# Autodesk Inventor assembly: 5 Barras Version 0
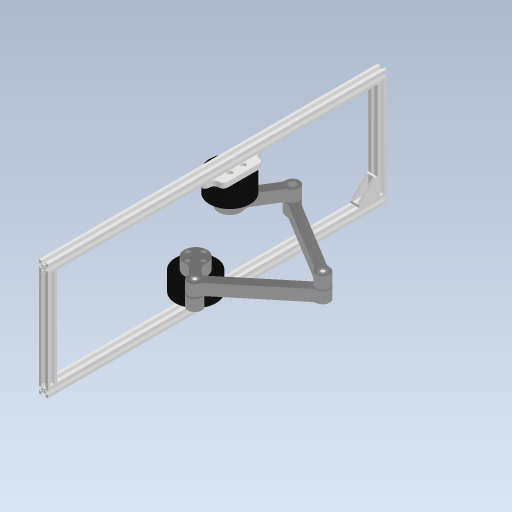
[picture p0: Inventor's stored thumbnail of the model, 512x512]
Saved by Autodesk Inventor 2024.2 (Build 282272000, 272)
## iProperties
Created: 2025-02-06
Part Number: 5 Barras Version 0
Document SubType Name: Assembly
Designer: jp.reyesf
Author: jp.reyesf
## Documents named in this file (18)
- C:\Users\jp.reyesf\Desktop\Master-Thesis\five_bar\assets\CAD\Robot\5 Barras Version 0.iam
- C:\Users\jp.reyesf\Desktop\Master-Thesis\five_bar\assets\CAD\Robot\Proximal Link 1.ipt
- C:\Users\jp.reyesf\Desktop\Master-Thesis\five_bar\assets\CAD\Robot\Distal Link 1.ipt
- C:\Users\jp.reyesf\Desktop\Master-Thesis\five_bar\assets\CAD\Robot\Distal Link 2.ipt
- C:\Users\jp.reyesf\Desktop\Master-Thesis\five_bar\assets\CAD\Robot\Proximal Link 2.ipt
- C:\Users\jp.reyesf\Desktop\Master-Thesis\five_bar\assets\CAD\Robot\Spacer.ipt
- C:\Users\jp.reyesf\Desktop\Master-Thesis\five_bar\assets\CAD\Robot\Bearing.ipt
- C:\Users\jp.reyesf\Desktop\Master-Thesis\five_bar\assets\CAD\Robot\Motor 1 Stator.ipt
- C:\Users\jp.reyesf\Desktop\Master-Thesis\five_bar\assets\CAD\Robot\Motor 1 Rotor.ipt
- C:\Users\jp.reyesf\Desktop\Master-Thesis\five_bar\assets\CAD\Robot\Motor 2 Stator.ipt
- C:\Users\jp.reyesf\Desktop\Master-Thesis\five_bar\assets\CAD\Robot\Motor 2 Rotor.ipt
- C:\Users\jp.reyesf\Desktop\Master-Thesis\five_bar\assets\CAD\Robot\separator.ipt
- C:\Users\jp.reyesf\Desktop\Master-Thesis\five_bar\assets\CAD\Robot\rod.ipt
- C:\Users\jp.reyesf\Desktop\Master-Thesis\five_bar\assets\CAD\Robot\Solid35.ipt
- C:\Users\jp.reyesf\Desktop\Master-Thesis\five_bar\assets\CAD\Robot\Solid37.ipt
- C:\Users\jp.reyesf\Desktop\Master-Thesis\five_bar\assets\CAD\Robot\Solid38.ipt
- C:\Users\jp.reyesf\Desktop\Master-Thesis\five_bar\assets\CAD\Robot\Spacer 2.ipt
- C:\Users\jp.reyesf\Desktop\Master-Thesis\five_bar\assets\CAD\Robot\Solid40.ipt
## Components (36 placed, 17 different names)
1. Proximal Link 1:1 — Mate:3, Mate:4, Mate:5, Mate:39, Mate:91, Mate:92
2. Distal Link 1:1 — Mate:39, Mate:43, Flush:4, Mate:93, Mate:94
3. Distal Link 2:1 — Mate:43, Mate:47, Flush:5, Mate:95, Mate:96
4. Proximal Link 2:1 — Mate:47, Mate:48, Mate:49, Flush:6
5. Motor 1 Stator:1 — Mate:1, Mate:2
6. Motor 1 Rotor:1 — Mate:1, Mate:2, Mate:3, Mate:4, Mate:5
7. Motor 2 Stator:1 — Mate:50, Mate:51
8. Motor 2 Rotor:1 — Mate:48, Mate:49, Mate:50, Mate:51
9. separator:1 — Mate:54, Mate:55, Mate:60, Mate:61
10. Spacer:4 — Mate:52, Mate:53, Mate:58, Mate:59
11. Bearing:8 — Mate:53, Mate:54, Mate:59, Mate:60
12. Bearing:9 — Mate:52, Mate:58, Flush:1, Mate:64, Mate:95, Mate:96
13. Bearing:12 — Mate:57, Mate:63, Flush:6
14. Bearing:13 — Mate:55, Mate:56, Mate:61, Mate:62
15. rod:1 — Flush:1, Mate:64
16. Solid35:1
17. Solid37:1
18. Solid38:1
19. Spacer 2:1 — Mate:56, Mate:57, Mate:62, Mate:63
20. Solid40:1
21. separator:2
22. Spacer:5
23. Bearing:14
24. Bearing:15 — Mate:91, Mate:92
25. Bearing:16 — Flush:4
26. Bearing:17
27. rod:2
28. Spacer 2:2
29. separator:3
30. Spacer:6
31. Bearing:18
32. Bearing:19 — Mate:93, Mate:94
33. Bearing:20 — Flush:5
34. Bearing:21
35. rod:3
36. Spacer 2:3
## Relationships (63: Mate 57, Flush 6)
- Mate:1: Motor 1 Stator:1 ↔ Motor 1 Rotor:1
- Mate:2: Motor 1 Stator:1 ↔ Motor 1 Rotor:1
- Mate:3: Proximal Link 1:1 ↔ Motor 1 Rotor:1
- Mate:4: Proximal Link 1:1 ↔ Motor 1 Rotor:1
- Mate:5: Proximal Link 1:1 ↔ Motor 1 Rotor:1
- Mate:39: Proximal Link 1:1 ↔ Distal Link 1:1
- Mate:43: Distal Link 1:1 ↔ Distal Link 2:1
- Mate:47: Distal Link 2:1 ↔ Proximal Link 2:1
- Mate:48: Proximal Link 2:1 ↔ Motor 2 Rotor:1
- Mate:49: Proximal Link 2:1 ↔ Motor 2 Rotor:1
- Mate:50: Motor 2 Stator:1 ↔ Motor 2 Rotor:1
- Mate:51: Motor 2 Stator:1 ↔ Motor 2 Rotor:1
- Mate:52: Spacer:4 ↔ Bearing:9
- Mate:53: Spacer:4 ↔ Bearing:8
- Mate:54 (0.1 mm): separator:1 ↔ Bearing:8
- Mate:55 (0.1 mm): separator:1 ↔ Bearing:13
- Mate:56: Bearing:13 ↔ Spacer 2:1
- Mate:57: Bearing:12 ↔ Spacer 2:1
- Mate:58: Spacer:4 ↔ Bearing:9
- Mate:59: Spacer:4 ↔ Bearing:8
- Mate:60: separator:1 ↔ Bearing:8
- Mate:61: separator:1 ↔ Bearing:13
- Mate:62: Bearing:13 ↔ Spacer 2:1
- Mate:63: Bearing:12 ↔ Spacer 2:1
- Flush:1: Bearing:9 ↔ rod:1
- Mate:64: Bearing:9 ↔ rod:1
- [Mate]: Spacer:5 ↔ Bearing:15
- [Mate]: Spacer:5 ↔ Bearing:14
- [Mate] (0.1 mm): separator:2 ↔ Bearing:14
- [Mate] (0.1 mm): separator:2 ↔ Bearing:17
- [Mate]: Bearing:17 ↔ Spacer 2:2
- [Mate]: Bearing:16 ↔ Spacer 2:2
- [Mate]: Spacer:5 ↔ Bearing:15
- [Mate]: Spacer:5 ↔ Bearing:14
- [Mate]: separator:2 ↔ Bearing:14
- [Mate]: separator:2 ↔ Bearing:17
- [Mate]: Bearing:17 ↔ Spacer 2:2
- [Mate]: Bearing:16 ↔ Spacer 2:2
- [Flush]: Bearing:15 ↔ rod:2
- [Mate]: Bearing:15 ↔ rod:2
- [Mate]: Spacer:6 ↔ Bearing:19
- [Mate]: Spacer:6 ↔ Bearing:18
- [Mate] (0.1 mm): separator:3 ↔ Bearing:18
- [Mate] (0.1 mm): separator:3 ↔ Bearing:21
- [Mate]: Bearing:21 ↔ Spacer 2:3
- [Mate]: Bearing:20 ↔ Spacer 2:3
- [Mate]: Spacer:6 ↔ Bearing:19
- [Mate]: Spacer:6 ↔ Bearing:18
- [Mate]: separator:3 ↔ Bearing:18
- [Mate]: separator:3 ↔ Bearing:21
- [Mate]: Bearing:21 ↔ Spacer 2:3
- [Mate]: Bearing:20 ↔ Spacer 2:3
- [Flush]: Bearing:19 ↔ rod:3
- [Mate]: Bearing:19 ↔ rod:3
- Mate:91: Proximal Link 1:1 ↔ Bearing:15
- Mate:92: Proximal Link 1:1 ↔ Bearing:15
- Flush:4: Distal Link 1:1 ↔ Bearing:16
- Mate:93: Distal Link 1:1 ↔ Bearing:19
- Mate:94: Distal Link 1:1 ↔ Bearing:19
- Flush:5: Distal Link 2:1 ↔ Bearing:20
- Mate:95: Distal Link 2:1 ↔ Bearing:9
- Mate:96: Distal Link 2:1 ↔ Bearing:9
- Flush:6: Proximal Link 2:1 ↔ Bearing:12
## Named parameters: d86_d72 = 0 mm, d87_d85 = 0 mm, d88_d73 = 0 mm, d89_d74 = 0.1 mm, d90_d75 = 0.1 mm, d91_d76 = 0 mm, d92_d77 = 0 mm, d93_d78 = 0 mm, d94_d79 = 0 mm, d95_d80 = 0 mm, d96_d81 = 0 mm, d97_d82 = 0 mm, d98_d83 = 0 mm, d99_d84 = 0 mm, d100_d72 = 0 mm, d101_d85 = 0 mm, d102_d73 = 0 mm, d103_d74 = 0.1 mm, d104_d75 = 0.1 mm, d105_d76 = 0 mm, d106_d77 = 0 mm, d107_d78 = 0 mm, d108_d79 = 0 mm, d109_d80 = 0 mm, d110_d81 = 0 mm, d111_d82 = 0 mm, d112_d83 = 0 mm, d113_d84 = 0 mm
